# Autodesk Inventor assembly: Assembly Leg
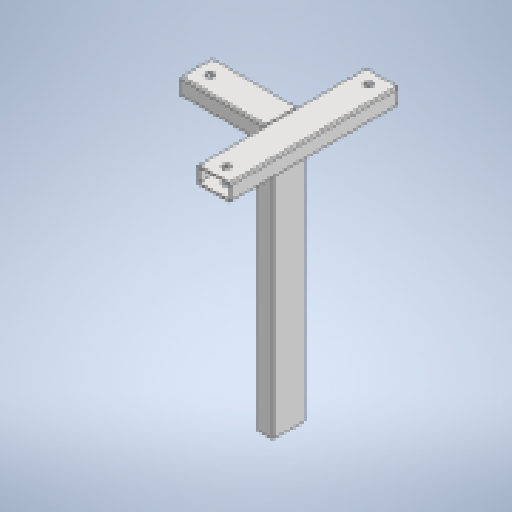
[picture p0: Inventor's stored thumbnail of the model, 512x512]
Saved by Autodesk Inventor 2026.2 (Build 302298000, 298)
## iProperties
Created: 2026-05-21
Part Number: Assembly Leg
Document SubType Name: Assembly
Designer: admin
Author: admin
## Documents named in this file (4)
- C:\Users\admin\Documents\Inventor\Debbed\Assembly Leg.iam
- C:\Users\admin\Documents\Inventor\Debbed\Leg tube 1.ipt
- C:\Users\admin\Documents\Inventor\Debbed\Leg tube 2.ipt
- C:\Users\admin\Documents\Inventor\Debbed\Leg tube 3.ipt
## Components (3 placed, 3 different names)
1. Leg tube 1:1
2. Leg tube 2:1
3. Leg tube 3:1
## Relationships (2: WeldJoint 2)
- [WeldJoint]: Leg tube 1:1 ↔ Leg tube 3:1
- [WeldJoint]: Leg tube 2:1 ↔ Leg tube 3:1
